# Autodesk Inventor assembly: BatteryUnit
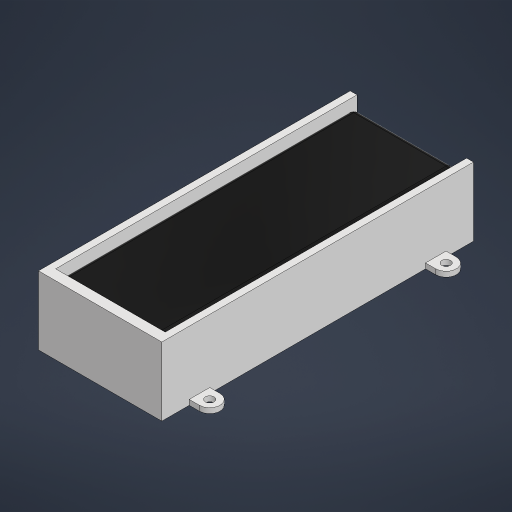
[picture p0: Inventor's stored thumbnail of the model, 512x512]
Saved by Autodesk Inventor 2024.2 (Build 282272000, 272)
## iProperties
Created: 2023-12-22
Part Number: BatteryUnit
Document SubType Name: Assembly
Designer: Hanaoka
Author: Hanaoka
## Documents named in this file (3)
- G:\共有ドライブ\reRo\05_個人\hanaoka\inventor\BatteryUnit\BatteryUnit.iam
- G:\共有ドライブ\reRo\05_個人\hanaoka\inventor\BatteryUnit\Battery_Noir3s1300mah.ipt
- G:\共有ドライブ\reRo\05_個人\hanaoka\inventor\BatteryUnit\BatteryCase.ipt
## Components (2 placed, 2 different names)
1. Battery_Noir3s1300mah:1 — メイト:3, メイト:4, メイト:5
2. BatteryCase:1 — フラッシュ:1, メイト:1, メイト:2, メイト:3, メイト:4, メイト:5
## Relationships (6: Mate 5, Flush 1)
- フラッシュ:1 [Flush]: BatteryCase:1
- メイト:1 [Mate]: BatteryCase:1
- メイト:2 [Mate] (-18 mm): BatteryCase:1
- メイト:3 [Mate]: Battery_Noir3s1300mah:1 ↔ BatteryCase:1
- メイト:4 [Mate]: Battery_Noir3s1300mah:1 ↔ BatteryCase:1
- メイト:5 [Mate] (1 mm): Battery_Noir3s1300mah:1 ↔ BatteryCase:1
